# Autodesk Inventor assembly: Autocollimator
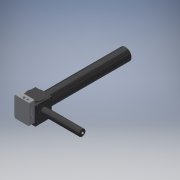
[picture p0: Inventor's stored thumbnail of the model, 180x180]
Saved by Autodesk Inventor 2018.3 (Build 223284000, 284)
## iProperties
Created: 2019-05-31
Part Number: Autocollimator
Document SubType Name: Assembly
Designer: 3esha
Author: 3esha
## Documents named in this file (18)
- E:\Autocollimator\Autocollimator2.iam
- E:\Autocollimator\BSW16-Step.ipt
- E:\Autocollimator\LA1131-B-Step.ipt
- E:\Autocollimator\LA1380-B-Step.ipt
- E:\Autocollimator\LB1C-Step.ipt
- E:\Autocollimator\LB3C-Step.ipt
- E:\Autocollimator\LB5CT1-Step.ipt
- E:\Autocollimator\LC6W-Step.ipt
- E:\Autocollimator\SM1L30-Step.ipt
- E:\Autocollimator\SM1L40-Step.ipt
- E:\Autocollimator\SM1RR-Step.ipt
- E:\Autocollimator\SM1SMA-Step.ipt
- E:\Autocollimator\SM2A6-Step.ipt
- E:\Autocollimator\SM2CP2-Step.ipt
- E:\Autocollimator\SM2E60-Step.ipt
- E:\Autocollimator\SM2L30-Step.ipt
- E:\Autocollimator\mask.ipt
- C:\Users\3esha\Downloads\TCE-1209-U.ipt
## Components (19 placed, 17 different names)
1. BSW16-Step:1 — Insert:1, Angle:2, Angle:3
2. LA1131-B-Step:1 — Rotational:1
3. LA1380-B-Step:1 — Insert:16
4. LB1C-Step:1 — Angle:4, Mate:2, Angle:5
5. LB3C-Step:1 — Mate:1, Angle:1, Angle:2, Insert:2
6. LB5CT1-Step:1 — Insert:1, Mate:1, Angle:1
7. LC6W-Step:1 — Insert:2, Angle:3, Angle:4, Mate:2, Insert:6, Insert:8, Insert:10, Insert:18, Angle:6
8. SM1L30-Step:1 — Insert:12, Insert:14
9. SM1L40-Step:1 — Insert:11, Insert:12, Insert:17, Rigid:1
10. SM1RR-Step:1 — Rotational:1
11. SM1SMA-Step:1 — Insert:14
12. SM2A6-Step:1 — Insert:10, Insert:11
13. SM2CP2-Step:1 — Insert:8
14. SM2E60-Step:1 — Insert:6, Mate:3
15. SM2L30-Step:1 — Insert:15, Insert:16
16. SM2E60-Step:2 — Insert:15, Mate:3
17. SM1RR-Step:2 — Rigid:1
18. mask:1 — Insert:17, Angle:5
19. TCE-1209-U:1 — Insert:18, Angle:6
## Relationships (23: Insert 12, Angle 6, Mate 3, RevoluteJoint 1, WeldJoint 1)
- Insert:1: BSW16-Step:1 ↔ LB5CT1-Step:1
- Mate:1: LB3C-Step:1 ↔ LB5CT1-Step:1
- Angle:1 (180 deg): LB3C-Step:1 ↔ LB5CT1-Step:1
- Angle:2 (0 deg): BSW16-Step:1 ↔ LB3C-Step:1
- Insert:2: LB3C-Step:1 ↔ LC6W-Step:1
- Angle:3 (45 deg): BSW16-Step:1 ↔ LC6W-Step:1
- Angle:4 (180 deg): LB1C-Step:1 ↔ LC6W-Step:1
- Mate:2: LB1C-Step:1 ↔ LC6W-Step:1
- Insert:6: LC6W-Step:1 ↔ SM2E60-Step:1
- Insert:8: LC6W-Step:1 ↔ SM2CP2-Step:1
- Insert:10: LC6W-Step:1 ↔ SM2A6-Step:1
- Insert:11: SM1L40-Step:1 ↔ SM2A6-Step:1
- Insert:12: SM1L30-Step:1 ↔ SM1L40-Step:1
- Insert:14: SM1L30-Step:1 ↔ SM1SMA-Step:1
- Insert:15: SM2L30-Step:1 ↔ SM2E60-Step:2
- Insert:16: LA1380-B-Step:1 ↔ SM2L30-Step:1
- Mate:3: SM2E60-Step:1 ↔ SM2E60-Step:2
- Rotational:1 [RevoluteJoint]: LA1131-B-Step:1 ↔ SM1RR-Step:1
- Insert:17 (50.8 mm): SM1L40-Step:1 ↔ mask:1
- Rigid:1 [WeldJoint]: SM1L40-Step:1 ↔ SM1RR-Step:2
- Angle:5 (0 deg): LB1C-Step:1 ↔ mask:1
- Insert:18: LC6W-Step:1 ↔ TCE-1209-U:1
- Angle:6 (0 deg): LC6W-Step:1 ↔ TCE-1209-U:1
